# Autodesk Inventor assembly: ASY NDM 11.023 перегородка рама 1 вертикал
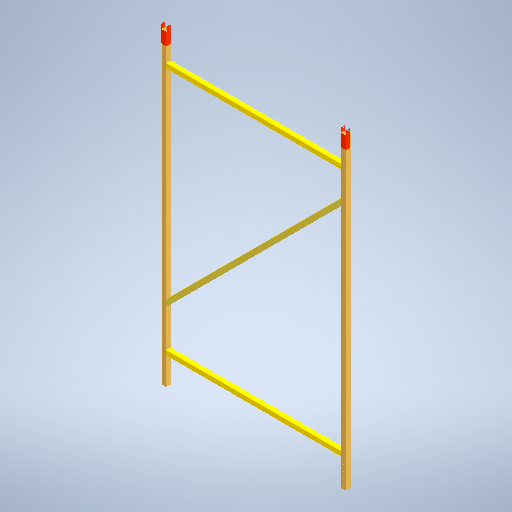
[picture p0: Inventor's stored thumbnail of the model, 512x512]
Saved by Autodesk Inventor 2025 (Build 290162010, 162A)
## iProperties
Created: 2024-06-11
Part Number: ASY NDM 11.023 перегородка рама 1 вертикал
Document SubType Name: Assembly
Designer: admin
Stock Number: NDM 11.023 перегородка рама 1 вертикал
Mass: 23442.7 g
Surface Area: 29483.2 cm^2
Volume: 2941.39 cm^3
Density: 7.96992 g/cm^3
_SolveAssemblyDoc: Frame Generator Solve Assembly
_Version: 25.0.0
Author: admin
Revision Number: 2
## Documents named in this file (4)
- C:\Users\user\YandexDisk\домашниий пк\Inventor\Nadyim\CAD\Перегородка\ASY NDM 11.023 перегородка рама 1 вертикал.iam
- C:\Users\user\YandexDisk\домашниий пк\Inventor\Nadyim\CAD\Перегородка\NDM 11.022 рама 1 вертикал.ipt
- C:\Users\user\YandexDisk\домашниий пк\Inventor\Nadyim\CAD\Перегородка\ASY NDM 11.023 перегородка рама 1 вертикал\Frame\Frame 1718103933196.iam
- C:\Users\user\YandexDisk\домашниий пк\Inventor\Nadyim\CAD\кронштейн\NDM 4.0.8 кронштейн связь 1.ipt
## Components (4 placed, 3 different names)
1. NDM 11.022 рама 1 вертикал:1 — Flush:1, Flush:2, Flush:3
2. Frame 1718103933196:1 [sub-assembly] — Mate:1, Mate:2, Flush:4, Mate:3, Flush:5, Mate:4
3. NDM 4.0.8 кронштейн связь 1:1 — Mate:1, Mate:2, Flush:4
4. NDM 4.0.8 кронштейн связь 1:2 — Mate:3, Flush:5, Mate:4
## Relationships (9: Flush 5, Mate 4)
- Flush:1: NDM 11.022 рама 1 вертикал:1
- Flush:2: NDM 11.022 рама 1 вертикал:1
- Flush:3: NDM 11.022 рама 1 вертикал:1
- Mate:1: Frame 1718103933196:1 ↔ NDM 4.0.8 кронштейн связь 1:1
- Mate:2: Frame 1718103933196:1 ↔ NDM 4.0.8 кронштейн связь 1:1
- Flush:4: Frame 1718103933196:1 ↔ NDM 4.0.8 кронштейн связь 1:1
- Mate:3: Frame 1718103933196:1 ↔ NDM 4.0.8 кронштейн связь 1:2
- Flush:5: Frame 1718103933196:1 ↔ NDM 4.0.8 кронштейн связь 1:2
- Mate:4: Frame 1718103933196:1 ↔ NDM 4.0.8 кронштейн связь 1:2
